# Autodesk Inventor assembly: Wheel And Drum
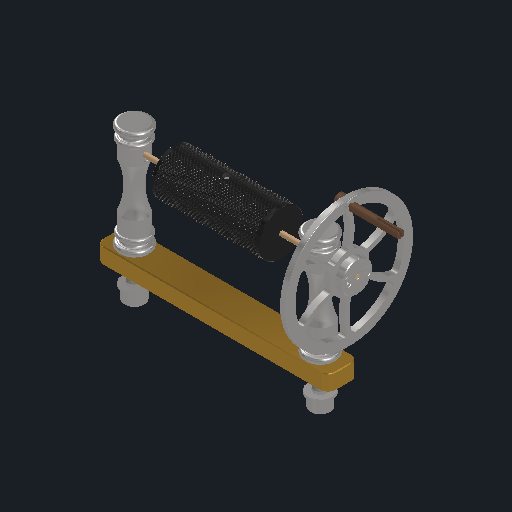
[picture p0: Inventor's stored thumbnail of the model, 512x512]
Saved by Autodesk Inventor 2027.1 (Build 311270010, 270A)
## iProperties
Created: 2025-09-16
Part Number: Wheel And Drum
Document SubType Name: Assembly
Designer: SD
Mass: 944.574 g
Surface Area: 463.098 cm^2
Volume: 117.441 cm^3
Density: 8.04297 g/cm^3
Project: Automatic Tea Steeping mechanism
BOM-Mass: 0.94457
BOM-Area: 0.046
Author: SD
Title: Wheel And Drum
## Documents named in this file (16)
- C:\Users\Gamer\Documents\Projects\Auto Tea Steeper\Public Version\Automatic Tea Steeper\CAD\Workspace\Wheel And Drum.iam
- C:\Users\Gamer\Documents\Projects\Auto Tea Steeper\Public Version\Automatic Tea Steeper\CAD\Workspace\Lower Arm Brass Plate - 3.ipt
- C:\Users\Gamer\Documents\Projects\Auto Tea Steeper\Public Version\Automatic Tea Steeper\CAD\Workspace\Ball Bearing-1.ipt
- C:\Users\Gamer\Documents\Projects\Auto Tea Steeper\Public Version\Automatic Tea Steeper\CAD\Workspace\Wheel Shaft 125mm.ipt
- C:\Users\Gamer\Documents\Projects\Auto Tea Steeper\Public Version\Automatic Tea Steeper\CAD\Workspace\Wheel.ipt
- C:\Users\Gamer\Documents\Projects\Auto Tea Steeper\Public Version\Automatic Tea Steeper\CAD\Workspace\Wheel Mounting Cap.ipt
- C:\Users\Gamer\Documents\Projects\Auto Tea Steeper\Public Version\Automatic Tea Steeper\CAD\Workspace\Drum.ipt
- C:\Users\Gamer\Documents\Projects\Auto Tea Steeper\Public Version\Automatic Tea Steeper\CAD\Workspace\Wheel Handle.ipt
- C:\Users\Gamer\Documents\Projects\Auto Tea Steeper\Public Version\Automatic Tea Steeper\CAD\Workspace\Hardware\Grub Screw 5x12mm.ipt
- C:\Users\Gamer\Documents\Projects\Auto Tea Steeper\Public Version\Automatic Tea Steeper\CAD\Workspace\Hardware\CSK Allen Key 3x8mm.ipt
- C:\Users\Gamer\Documents\Projects\Auto Tea Steeper\Public Version\Automatic Tea Steeper\CAD\Workspace\Hardware\Grub Screw 3x8mm.ipt
- C:\Users\Gamer\Documents\Projects\Auto Tea Steeper\Public Version\Automatic Tea Steeper\CAD\Workspace\Hardware\Allen Key 8x40mm.ipt
- C:\Users\Gamer\Documents\Projects\Auto Tea Steeper\Public Version\Automatic Tea Steeper\CAD\Workspace\Wheel Shaft Pillar.ipt
- C:\Users\Gamer\Documents\Projects\Auto Tea Steeper\Public Version\Automatic Tea Steeper\CAD\Workspace\Wheel Shaft Pillar - 2.ipt
- C:\Users\Gamer\Documents\Projects\Auto Tea Steeper\Public Version\Automatic Tea Steeper\CAD\Workspace\Hardware\8mm Washer.ipt
- C:\Users\Gamer\Documents\Projects\Auto Tea Steeper\Public Version\Automatic Tea Steeper\CAD\Workspace\Hardware\4mm E Clip.ipt
## Components (20 placed, 14 different names)
1. Lower Arm Brass Plate - 3:1 — Mate:18, Flush:3, Mate:29, Mate:31, Mate:32, Mate:35, Angle:2, Mate:41, Angle:3
2. 683ZZ Ball Bearing:1 — Mate:38, Mate:39
3. 683ZZ Ball Bearing:2 — Mate:11, Mate:42, Mate:43
4. 683ZZ Ball Bearing:3 — Mate:36, Mate:37
5. Wheel Shaft 125mm:1 — Mate:11, Mate:13, Mate:15, Flush:1, Mate:20, Mate:24
6. Wheel:1 — Mate:13, Mate:16, Mate:17, Mate:18, Mate:33, Mate:48, Mate:49
7. Wheel Mounting Cap:1 — Mate:16, Mate:17, Flush:1, Mate:21, Flush:4, Mate:22, Flush:5, Mate:23
8. Drum:1 — Mate:15, Flush:3, Mate:19
9. Wheel Handle:1 — Mate:48, Mate:49, Mate:50, Mate:51
10. ISO 4026 M3 x 3:1 — Mate:19, Mate:20
11. CSK Allen Key 3x8mm:1 — Mate:21, Flush:4
12. CSK Allen Key 3x8mm:2 — Mate:22, Flush:5, Mate:33
13. ISO 4026 M3 x 3:2 — Mate:23, Mate:24
14. Allen Key 8x40mm:1 — Mate:29, Mate:34, Flush:6, Mate:45, Mate:46
15. Allen Key 8x40mm:2 — Mate:31, Mate:32, Mate:40, Flush:6, Mate:44, Mate:47
16. Wheel Shaft Pillar:1 — Mate:34, Mate:35, Angle:2, Mate:36, Mate:37, Mate:38, Mate:39
17. Wheel Shaft Pillar - 2:1 — Mate:40, Mate:41, Angle:3, Mate:42, Mate:43
18. ISO 7089 8:1 — Mate:44, Mate:47
19. ISO 7089 8:2 — Mate:45, Mate:46
20. 4mm E Clip:1 — Mate:50, Mate:51
## Relationships (41: Mate 34, Flush 5, Angle 2)
- Mate:11: 683ZZ Ball Bearing:2 ↔ Wheel Shaft 125mm:1
- Mate:13: Wheel Shaft 125mm:1 ↔ Wheel:1
- Mate:15: Wheel Shaft 125mm:1 ↔ Drum:1
- Mate:16: Wheel:1 ↔ Wheel Mounting Cap:1
- Mate:17: Wheel:1 ↔ Wheel Mounting Cap:1
- Flush:1: Wheel Shaft 125mm:1 ↔ Wheel Mounting Cap:1
- Mate:18: Lower Arm Brass Plate - 3:1 ↔ Wheel:1
- Flush:3: Lower Arm Brass Plate - 3:1 ↔ Drum:1
- Mate:19: Drum:1 ↔ ISO 4026 M3 x 3:1
- Mate:20: Wheel Shaft 125mm:1 ↔ ISO 4026 M3 x 3:1
- Mate:21: Wheel Mounting Cap:1 ↔ CSK Allen Key 3x8mm:1
- Flush:4: Wheel Mounting Cap:1 ↔ CSK Allen Key 3x8mm:1
- Mate:22: Wheel Mounting Cap:1 ↔ CSK Allen Key 3x8mm:2
- Flush:5: Wheel Mounting Cap:1 ↔ CSK Allen Key 3x8mm:2
- Mate:23: Wheel Mounting Cap:1 ↔ ISO 4026 M3 x 3:2
- Mate:24: Wheel Shaft 125mm:1 ↔ ISO 4026 M3 x 3:2
- Mate:29: Lower Arm Brass Plate - 3:1 ↔ Allen Key 8x40mm:1
- Mate:31: Lower Arm Brass Plate - 3:1 ↔ Allen Key 8x40mm:2
- Mate:32 (11.5 mm): Lower Arm Brass Plate - 3:1 ↔ Allen Key 8x40mm:2
- Mate:33: Wheel:1 ↔ CSK Allen Key 3x8mm:2
- Mate:34: Allen Key 8x40mm:1 ↔ Wheel Shaft Pillar:1
- Mate:35: Lower Arm Brass Plate - 3:1 ↔ Wheel Shaft Pillar:1
- Angle:2 (0 deg): Lower Arm Brass Plate - 3:1 ↔ Wheel Shaft Pillar:1
- Mate:36: 683ZZ Ball Bearing:3 ↔ Wheel Shaft Pillar:1
- Mate:37: 683ZZ Ball Bearing:3 ↔ Wheel Shaft Pillar:1
- Mate:38: 683ZZ Ball Bearing:1 ↔ Wheel Shaft Pillar:1
- Mate:39: 683ZZ Ball Bearing:1 ↔ Wheel Shaft Pillar:1
- Mate:40: Allen Key 8x40mm:2 ↔ Wheel Shaft Pillar - 2:1
- Mate:41: Lower Arm Brass Plate - 3:1 ↔ Wheel Shaft Pillar - 2:1
- Angle:3 (0 deg): Lower Arm Brass Plate - 3:1 ↔ Wheel Shaft Pillar - 2:1
- Mate:42: 683ZZ Ball Bearing:2 ↔ Wheel Shaft Pillar - 2:1
- Mate:43: 683ZZ Ball Bearing:2 ↔ Wheel Shaft Pillar - 2:1
- Flush:6: Allen Key 8x40mm:1 ↔ Allen Key 8x40mm:2
- Mate:44: Allen Key 8x40mm:2 ↔ ISO 7089 8:1
- Mate:45: Allen Key 8x40mm:1 ↔ ISO 7089 8:2
- Mate:46: Allen Key 8x40mm:1 ↔ ISO 7089 8:2
- Mate:47: Allen Key 8x40mm:2 ↔ ISO 7089 8:1
- Mate:48: Wheel:1 ↔ Wheel Handle:1
- Mate:49: Wheel:1 ↔ Wheel Handle:1
- Mate:50: Wheel Handle:1 ↔ 4mm E Clip:1
- Mate:51: Wheel Handle:1 ↔ 4mm E Clip:1
